# Autodesk Inventor assembly: complete
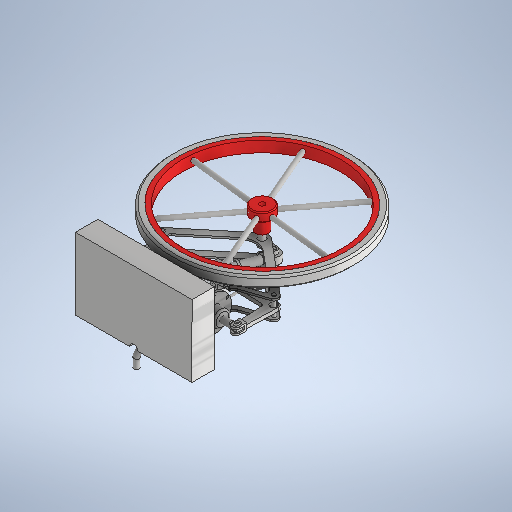
[picture p0: Inventor's stored thumbnail of the model, 512x512]
Saved by Autodesk Inventor 2025.1 (Build 291241000, 241)
## iProperties
Created: 2024-09-14
Part Number: complete
Document SubType Name: Assembly
Designer: ffogue
Author: ffogue
## Documents named in this file (27)
- C:\Users\ffogue\Documents\Inventor\Single cylinder Steam Engine\complete.iam
- C:\Users\ffogue\Documents\Inventor\Single cylinder Steam Engine\block.ipt
- C:\Users\ffogue\Documents\Inventor\Single cylinder Steam Engine\02.ipt
- C:\Users\ffogue\Documents\Inventor\Single cylinder Steam Engine\06.ipt
- C:\Users\ffogue\Documents\Inventor\Single cylinder Steam Engine\16.ipt
- C:\Users\ffogue\Documents\Inventor\Single cylinder Steam Engine\15.ipt
- C:\Users\ffogue\Documents\Inventor\Single cylinder Steam Engine\17.ipt
- C:\Users\ffogue\Documents\Inventor\Single cylinder Steam Engine\14.iam
- C:\Users\ffogue\Documents\Inventor\Single cylinder Steam Engine\11.iam
- C:\Users\ffogue\Documents\Inventor\Single cylinder Steam Engine\24.iam
- C:\Users\ffogue\Documents\Inventor\Single cylinder Steam Engine\25.iam
- C:\Users\ffogue\Documents\Inventor\Single cylinder Steam Engine\08.ipt
- C:\Users\ffogue\Documents\Inventor\Single cylinder Steam Engine\9.ipt
- C:\Users\ffogue\Documents\Inventor\Single cylinder Steam Engine\10.ipt
- C:\Users\ffogue\Documents\Inventor\Single cylinder Steam Engine\10.2.ipt
- C:\Users\ffogue\Documents\Inventor\Single cylinder Steam Engine\07.ipt
- C:\Users\ffogue\Documents\Inventor\Single cylinder Steam Engine\01.ipt
- C:\Users\ffogue\Documents\Inventor\Single cylinder Steam Engine\fitting.ipt
- C:\Users\ffogue\Documents\Inventor\Single cylinder Steam Engine\9.1.ipt
- C:\Users\ffogue\Documents\Inventor\Single cylinder Steam Engine\13.iam
- C:\Users\ffogue\Documents\Inventor\Single cylinder Steam Engine\12.iam
- C:\Users\ffogue\Documents\Inventor\Single cylinder Steam Engine\19.iam
- C:\Users\ffogue\Documents\Inventor\Single cylinder Steam Engine\21.iam
- C:\Users\ffogue\Documents\Inventor\Single cylinder Steam Engine\20.iam
- C:\Users\ffogue\Documents\Inventor\Single cylinder Steam Engine\22.iam
- C:\Users\ffogue\Documents\Inventor\Single cylinder Steam Engine\18.ipt
- C:\Users\ffogue\Documents\Inventor\Single cylinder Steam Engine\13 s.ipt
## Components (35 placed, 26 different names)
1. block:1 — Flush:1, Mate:1, Flush:4, Angle:1
2. 02:1 — Flush:1, Mate:1, Mate:2, Insert:1
3. 06:1 — Mate:2, Insert:1, Mate:3, Insert:2, Mate:6, Mate:7, Insert:5, Mate:9, Mate:10, Insert:6, Mate:21, Mate:22, Insert:11, Insert:12, Mate:26, Insert:15, Mate:27, Insert:16
4. 16:1 — Mate:3, Insert:2, Mate:4, Insert:3
5. 15:1 — Mate:4, Insert:3, Mate:5, Insert:4, Mate:12, Insert:7, Mate:13, Insert:8, Mate:56
6. 17:1 — Mate:5, Insert:4
7. 14:1 [sub-assembly] — Mate:6, Mate:7, Insert:5, Mate:8
8. 11:1 [sub-assembly] — Mate:8, Mate:20, Mate:48, Rotational:2, Mate:61
9. 11:2 [sub-assembly] — Mate:11, Mate:50, Rotational:1, Mate:62
10. 14:2 [sub-assembly] — Mate:9, Mate:10, Insert:6, Mate:11
11. 24:1 [sub-assembly] — Mate:12, Insert:7
12. 25:1 [sub-assembly] — Mate:13, Insert:8
13. 08:1 — Mate:14, Mate:23, Mate:24, Cylindrical:3, Mate:47, Mate:49, Insert:17
14. 9:1 — Mate:14, Insert:17, Mate:51, Insert:18
15. 10:1 — Mate:15, Insert:9, Mate:20, Mate:32, Mate:33, Mate:35, Mate:36, Mate:48, Rotational:2, Flush:6
16. 10.2:1 — Mate:15, Insert:9, Mate:47, Flush:8
17. 10:2 — Mate:49, Mate:50, Rotational:1, Flush:7, Mate:63
18. 07:1 — Mate:21, Insert:12, Mate:23, Cylindrical:3
19. 07:2 — Mate:22, Insert:11, Mate:24
20. 01:1 — Mate:26, Insert:15, Flush:3, Mate:52, Insert:20
21. 01:2 — Mate:27, Insert:16, Mate:30, Mate:31
22. fitting:1 — Mate:30, Mate:31, Flush:3, Mate:34, Mate:37, Mate:40, Mate:45
23. 9.1:1 — Mate:32, Mate:33, Mate:36
24. 9.1:2 — Mate:37, Mate:45
25. 13:1 [sub-assembly] — Mate:51, Insert:18, Mate:53, Insert:19
26. 12:1 [sub-assembly] — Mate:52, Mate:53, Insert:19, Mate:55, Mate:60, Rotation:2, Mate:64, Flush:9
27. 19:1 [sub-assembly] — Mate:54, Mate:56, Mate:59, Flush:5
28. 21:1 [sub-assembly] — Mate:54, Mate:57, Insert:21
29. 20:1 [sub-assembly] — Mate:55, Insert:20, Mate:57, Insert:21, Rotation:1
30. 18:1 — Mate:59, Flush:5
31. 22:1 [sub-assembly] — Mate:60, Angle:1, Rotation:1, Rotation:2
32. 10.2:2 — Mate:61, Flush:6
33. 10.2:3 — Mate:62, Flush:7
34. 10.2:4 — Mate:63, Flush:8
35. 13 s:1 — Mate:64, Flush:9
## Relationships (81: Mate 49, Insert 18, Flush 8, RevoluteJoint 2, RelateRotation 2, CylindricalJoint 1, Angle 1)
- Flush:1 (15 mm): block:1 ↔ 02:1
- Mate:1: block:1 ↔ 02:1
- Mate:2: 02:1 ↔ 06:1
- Insert:1: 02:1 ↔ 06:1
- Mate:3: 06:1 ↔ 16:1
- Insert:2: 06:1 ↔ 16:1
- Mate:4: 16:1 ↔ 15:1
- Insert:3: 16:1 ↔ 15:1
- Mate:5: 15:1 ↔ 17:1
- Insert:4: 15:1 ↔ 17:1
- Mate:6: 06:1 ↔ 14:1
- Mate:7: 06:1 ↔ 14:1
- Insert:5: 06:1 ↔ 14:1
- Mate:8: 14:1 ↔ 11:1
- Mate:9: 06:1 ↔ 14:2
- Mate:10: 06:1 ↔ 14:2
- Insert:6: 06:1 ↔ 14:2
- Mate:11: 11:2 ↔ 14:2
- Mate:12: 15:1 ↔ 24:1
- Insert:7: 15:1 ↔ 24:1
- Mate:13: 15:1 ↔ 25:1
- Insert:8: 15:1 ↔ 25:1
- Mate:14: 08:1 ↔ 9:1
- Mate:15: 10:1 ↔ 10.2:1
- Insert:9 (-8 mm): 10:1 ↔ 10.2:1
- Mate:20: 11:1 ↔ 10:1
- Mate:21: 06:1 ↔ 07:1
- Mate:22: 06:1 ↔ 07:2
- Insert:11: 06:1 ↔ 07:2
- Insert:12: 06:1 ↔ 07:1
- Mate:23: 08:1 ↔ 07:1
- Mate:24: 08:1 ↔ 07:2
- Cylindrical:3: 08:1 ↔ 07:1
- Mate:26: 06:1 ↔ 01:1
- Insert:15: 06:1 ↔ 01:1
- Mate:27: 06:1 ↔ 01:2
- Insert:16: 06:1 ↔ 01:2
- Mate:30: 01:2 ↔ fitting:1
- Mate:31: 01:2 ↔ fitting:1
- Flush:3 (-1 mm): 01:1 ↔ fitting:1
- Mate:32: 10:1 ↔ 9.1:1
- Mate:33: 10:1 ↔ 9.1:1
- Mate:34: fitting:1
- Mate:35: 10:1
- Mate:36: 10:1 ↔ 9.1:1
- Mate:37: fitting:1 ↔ 9.1:2
- Mate:40: fitting:1
- Mate:45: fitting:1 ↔ 9.1:2
- Mate:47: 08:1 ↔ 10.2:1
- Mate:48: 11:1 ↔ 10:1
- Mate:49: 08:1 ↔ 10:2
- Mate:50: 11:2 ↔ 10:2
- Rotational:1 [RevoluteJoint] (-2 mm): 11:2 ↔ 10:2
- Rotational:2 [RevoluteJoint] (2 mm): 11:1 ↔ 10:1
- Insert:17: 08:1 ↔ 9:1
- Mate:51: 9:1 ↔ 13:1
- Insert:18: 9:1 ↔ 13:1
- Mate:52: 01:1 ↔ 12:1
- Mate:53: 13:1 ↔ 12:1
- Insert:19: 13:1 ↔ 12:1
- Flush:4: block:1
- Mate:54: 19:1 ↔ 21:1
- Mate:55: 12:1 ↔ 20:1
- Insert:20 (4.25 mm): 01:1 ↔ 20:1
- Mate:56: 15:1 ↔ 19:1
- Mate:57: 21:1 ↔ 20:1
- Insert:21: 21:1 ↔ 20:1
- Mate:59: 19:1 ↔ 18:1
- Flush:5: 19:1 ↔ 18:1
- Mate:60: 12:1 ↔ 22:1
- Angle:1 (0 deg): block:1 ↔ 22:1
- Rotation:1 [RelateRotation] (1 ul): 20:1 ↔ 22:1
- Rotation:2 [RelateRotation] (1 ul): 12:1 ↔ 22:1
- Mate:61: 11:1 ↔ 10.2:2
- Flush:6 (-2 mm): 10:1 ↔ 10.2:2
- Mate:62: 11:2 ↔ 10.2:3
- Flush:7 (-2 mm): 10:2 ↔ 10.2:3
- Mate:63: 10:2 ↔ 10.2:4
- Flush:8: 10.2:1 ↔ 10.2:4
- Mate:64: 12:1 ↔ 13 s:1
- Flush:9: 12:1 ↔ 13 s:1
